# Autodesk Inventor assembly: outsideCover
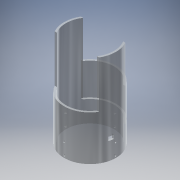
[picture p0: Inventor's stored thumbnail of the model, 180x180]
Saved by Autodesk Inventor 2016 (Build 200138000, 138)
## iProperties
Created: 2016-11-13
Part Number: outsideCover
Material: 一般
Document SubType Name: Assembly
Designer: Daisuke
Author: Daisuke
## Documents named in this file (3)
- C:\Users\Daisuke\Documents\GitHub\CAD\Hand\ver2\outsideCover.iam
- C:\Users\Daisuke\Documents\GitHub\CAD\Hand\ver2\outsideCover1.ipt
- C:\Users\Daisuke\Documents\GitHub\CAD\Hand\ver2\outsideCover2.ipt
## Components (2 placed, 2 different names)
1. outsideCover1:1 — 挿入:1, メイト:1
2. outsideCover2:1 — 挿入:1, メイト:1
## Relationships (2: Insert 1, Mate 1)
- 挿入:1 [Insert]: outsideCover1:1 ↔ outsideCover2:1
- メイト:1 [Mate]: outsideCover1:1 ↔ outsideCover2:1
